# Autodesk Inventor assembly: bloc_codeur
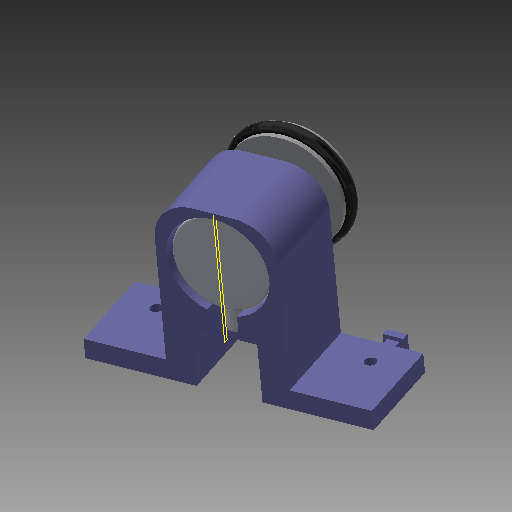
[picture p0: Inventor's stored thumbnail of the model, 512x512]
Saved by Autodesk Inventor 2019 (Build 230136000, 136)
## iProperties
Created: 2017-12-27
Part Number: bloc_codeur
Document SubType Name: Assembly
Designer: franc
Mass: 28.9449 g
Surface Area: 195.451 cm^2
Volume: 27.4271 cm^3
Density: 1.05534 g/cm^3
Author: franc
## Documents named in this file (5)
- C:\Users\franc\Desktop\EsialRobotik\Mecanique\base_roulante\bloc_codeur.iam
- C:\Users\franc\Desktop\EsialRobotik\Mecanique\base_roulante\composants\codeur_kubler_05.2400_11X2_XXXX.ipt
- C:\Users\franc\Desktop\EsialRobotik\Mecanique\base_roulante\composants\support_codeur.ipt
- C:\Users\franc\Desktop\EsialRobotik\Mecanique\base_roulante\composants\Roue de mesure Scancon 100 mm -ID64.ipt
- C:\Users\franc\Desktop\EsialRobotik\Mecanique\Content Center Files\R2017\fr-FR\CNS 4355\CNS 4355 - M 3 x 5.ipt
## Components (6 placed, 4 different names)
1. codeur_kubler_05.2400_11X2_XXXX:1 — Placage:2, Placage:3, Placage:4, Placage:5, Placage:6, Placage:7, Placage:8, Placage:9
2. support_codeur:1 — Placage:3, Placage:5, Placage:6, Placage:10, Placage:11, Placage:12
3. Roue de mesure Scancon 100 mm -ID64:1 — Placage:2, Placage:4
4. CNS 4355 M 3 x 5:1 — Placage:8, Placage:12
5. CNS 4355 M 3 x 5:3 — Placage:9, Placage:11
6. CNS 4355 M 3 x 5:4 — Placage:7, Placage:10
## Relationships (11: Mate 11)
- Placage:2 [Mate]: codeur_kubler_05.2400_11X2_XXXX:1 ↔ Roue de mesure Scancon 100 mm -ID64:1
- Placage:3 [Mate]: codeur_kubler_05.2400_11X2_XXXX:1 ↔ support_codeur:1
- Placage:4 [Mate] (1 mm): codeur_kubler_05.2400_11X2_XXXX:1 ↔ Roue de mesure Scancon 100 mm -ID64:1
- Placage:5 [Mate]: codeur_kubler_05.2400_11X2_XXXX:1 ↔ support_codeur:1
- Placage:6 [Mate]: codeur_kubler_05.2400_11X2_XXXX:1 ↔ support_codeur:1
- Placage:7 [Mate]: codeur_kubler_05.2400_11X2_XXXX:1 ↔ CNS 4355 M 3 x 5:4
- Placage:8 [Mate]: codeur_kubler_05.2400_11X2_XXXX:1 ↔ CNS 4355 M 3 x 5:1
- Placage:9 [Mate]: codeur_kubler_05.2400_11X2_XXXX:1 ↔ CNS 4355 M 3 x 5:3
- Placage:10 [Mate]: support_codeur:1 ↔ CNS 4355 M 3 x 5:4
- Placage:11 [Mate]: support_codeur:1 ↔ CNS 4355 M 3 x 5:3
- Placage:12 [Mate]: support_codeur:1 ↔ CNS 4355 M 3 x 5:1
